# Autodesk Inventor assembly: Ensemble_Attache_Bandoulière
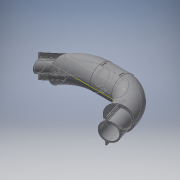
[picture p0: Inventor's stored thumbnail of the model, 180x180]
Saved by Autodesk Inventor 2016 (Build 200138000, 138)
## iProperties
Created: 2016-05-08
Part Number: Ensemble_Attache_Bandoulière
Material: Générique
Document SubType Name: Assembly
Designer: Ropert
Author: Ropert
## Documents named in this file (4)
- C:\Users\Ropert\Documents\LISAA\AD4\PFE\PROJET\pièces 3D\3\Ensemble_Attache_Bandoulière.iam
- C:\Users\Ropert\Documents\LISAA\AD4\PFE\PROJET\pièces 3D\3\goulot.ipt
- C:\Users\Ropert\Documents\LISAA\AD4\PFE\PROJET\pièces 3D\3\pièce intermédiaire.ipt
- C:\Users\Ropert\Documents\LISAA\AD4\PFE\PROJET\pièces 3D\3\passage robinet.ipt
## Components (3 placed, 3 different names)
1. goulot:1 — Affleurement:1, Placage:1, Placage:2, Affleurement:3
2. pièce intermédiaire:1 — Affleurement:1, Affleurement:2
3. passage robinet:1 — Affleurement:2, Placage:1, Placage:2, Affleurement:3
## Relationships (5: Flush 3, Mate 2)
- Affleurement:1 [Flush]: goulot:1 ↔ pièce intermédiaire:1
- Affleurement:2 [Flush]: pièce intermédiaire:1 ↔ passage robinet:1
- Placage:1 [Mate]: goulot:1 ↔ passage robinet:1
- Placage:2 [Mate]: goulot:1 ↔ passage robinet:1
- Affleurement:3 [Flush]: goulot:1 ↔ passage robinet:1
